# Autodesk Inventor assembly: ASY PNS 1200 right module
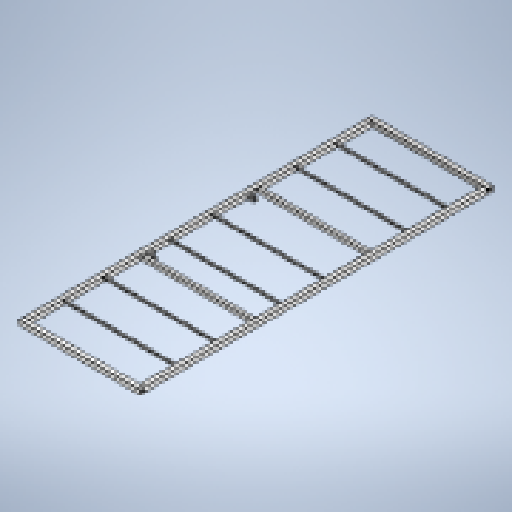
[picture p0: Inventor's stored thumbnail of the model, 512x512]
Saved by Autodesk Inventor 2025.3 (Build 293356030, 356C)
## iProperties
Created: 2025-03-25
Part Number: ASY PNS 1200 right module
Document SubType Name: Assembly
Designer: user
Author: user
## Documents named in this file (17)
- C:\Users\admin\Yandex.Disk\home pc\Inventor\PNS2-Panaevsk\ASY PNS 1200 right module.iam
- C:\Users\admin\Yandex.Disk\home pc\Inventor\PNS2-Panaevsk\ASY PNS 1220 frame right floor.iam
- C:\Users\admin\Yandex.Disk\home pc\Inventor\PNS2-Panaevsk\ASY PNS 1240 frame featheredge.iam
- C:\Users\admin\Yandex.Disk\home pc\Inventor\PNS2-Panaevsk\ASY PNS 1130 frame featheredge.iam
- C:\Users\admin\Yandex.Disk\home pc\Inventor\PNS2-Panaevsk\PNS-0261 Upper beam.ipt
- C:\Users\admin\Yandex.Disk\home pc\Inventor\PNS2-Panaevsk\PNS-0262 middle pillar.ipt
- C:\Users\admin\Yandex.Disk\home pc\Inventor\PNS2-Panaevsk\PNS-0262 cross beam.ipt
- C:\Users\admin\Yandex.Disk\home pc\Inventor\PNS2-Panaevsk\PNS-071 stretch ring.ipt
- C:\Users\admin\Yandex.Disk\home pc\Inventor\PNS2-Panaevsk\PNS-0310 strench.ipt
- C:\Users\admin\Yandex.Disk\home pc\Inventor\PNS2-Panaevsk\PNS-0810 floor ring.ipt
- C:\Users\admin\Yandex.Disk\home pc\Inventor\PNS2-Panaevsk\PNS-0812 floor ring  strengthen.ipt
- C:\Users\admin\Yandex.Disk\home pc\Inventor\PNS2-Panaevsk\PNS-073 stretch tear.ipt
- C:\Users\admin\Yandex.Disk\home pc\Inventor\PNS2-Panaevsk\PNS-0872 roof ring.ipt
- C:\Users\admin\Yandex.Disk\home pc\Inventor\PNS2-Panaevsk\PNS-077 stretch plate.ipt
- C:\Users\admin\Yandex.Disk\home pc\Inventor\PNS2-Panaevsk\PNS-0263 cross beam3.ipt
- C:\Users\admin\Yandex.Disk\home pc\Inventor\PNS2-Panaevsk\PNS-slings.ipt
- C:\Users\admin\Yandex.Disk\home pc\Inventor\PNS2-Panaevsk\PNS-slings_2.ipt
## Components (40 placed, 16 different names)
1. ASY PNS 1220 frame right floor:1 [sub-assembly] — Rigid:3, Mate:38, Flush:9, Mate:42, Mate:44, Mate:64, Mate:65, Mate:69
2. ASY PNS 1240 frame featheredge:1 [sub-assembly] — Rigid:4, Rigid:5, Rigid:6, Rigid:7, Mate:41, Mate:68
3. ASY PNS 1130 frame featheredge:1 [sub-assembly] — Rigid:3, Rigid:8, Rigid:9, Mate:37, Mate:40, Mate:55, Mate:56
4. PNS-0261 Upper beam:1 — Rigid:4, Mate:5, Flush:3, Mate:6, Flush:4, Mate:26, Mate:27, Tangent:4, Mate:35, Flush:8, Mate:39, Mate:46, Mate:49, Mate:50, Mate:51, Mate:52, Mate:53, Mate:54, Flush:17, Flush:18, Flush:19, Flush:20, Flush:21, Flush:22, Mate:61, Mate:63, Mate:67, Mate:77, Flush:73
5. PNS-0261 Upper beam:2 — Rigid:5, Mate:73, Mate:74, Mate:75, Mate:76
6. PNS-0262 middle pillar:1 — Rigid:6, Mate:43, Mate:66
7. PNS-0262 middle pillar:2 — Rigid:7, Flush:16
8. PNS-0262 middle pillar:3 — Rigid:8, Mate:36, Mate:45
9. PNS-0262 middle pillar:4 — Rigid:9, Flush:23
10. PNS-0262 cross beam:1 — Mate:6, Flush:4, Flush:23, Mate:57, Mate:58
11. PNS-0262 cross beam:2 — Mate:5, Flush:3, Flush:16, Mate:59, Mate:60
12. PNS-071 stretch ring:1 — Flush:12, Mate:66, Mate:67
13. PNS-071 stretch ring:2 — Flush:14, Mate:68, Mate:69
14. PNS-0310 strench:1
15. PNS-071 stretch ring:3 — Rotational:1, Mate:35, Mate:36, Flush:8, Flush:11, Flush:12
16. PNS-071 stretch ring:4 — Mate:37, Mate:38, Flush:9, Flush:10, Flush:14, Flush:15
17. PNS-0310 strench:2 — Mate:16, Tangent:3, Mate:17, Mate:21
18. PNS-0810 floor ring:2 — Mate:62, Flush:64, Flush:65, Mate:64
19. PNS-073 stretch tear:1 — Rotational:1, Mate:16, Tangent:3, Mate:17, Flush:6, Flush:7
20. PNS-073 stretch tear:2 — Mate:21, Flush:6, Flush:7
21. PNS-0812 floor ring  strengthen:2 — Mate:61, Mate:62, Flush:64, Flush:65, Mate:63, Flush:72
22. PNS-0810 floor ring:3 — Mate:28, Tangent:4
23. PNS-0812 floor ring  strengthen:3 — Mate:26, Mate:27, Mate:28, Mate:65, Flush:71
24. PNS-0872 roof ring:1 — Mate:77, Flush:73
25. PNS-077 stretch plate:1 — Mate:39, Mate:40, Flush:10
26. PNS-077 stretch plate:2 — Mate:44, Mate:45, Flush:11, Flush:13
27. PNS-077 stretch plate:3 — Mate:42, Mate:43, Flush:13
28. PNS-077 stretch plate:4 — Mate:41, Flush:15, Mate:46
29. PNS-0263 cross beam3:1 — Mate:49, Flush:22, Mate:55
30. PNS-0263 cross beam3:2 — Mate:50, Flush:21, Mate:56
31. PNS-0263 cross beam3:3 — Mate:51, Flush:20, Mate:57
32. PNS-0263 cross beam3:4 — Mate:52, Flush:19, Mate:58
33. PNS-0263 cross beam3:5 — Mate:53, Flush:18, Mate:59
34. PNS-0263 cross beam3:6 — Mate:54, Flush:17, Mate:60
35. PNS-slings:1
36. PNS-slings_2:1 — Mate:70
37. PNS-0810 floor ring:4
38. PNS-0812 floor ring  strengthen:4 — Mate:74, Mate:75, Flush:72
39. PNS-0810 floor ring:5
40. PNS-0812 floor ring  strengthen:5 — Mate:73, Mate:76, Flush:71
## Relationships (93: Mate 51, Flush 31, WeldJoint 8, Tangent 2, RevoluteJoint 1)
- [WeldJoint]: ASY PNS 1220 frame right floor:1 ↔ ASY PNS 1240 frame featheredge:1
- Rigid:3 [WeldJoint]: ASY PNS 1220 frame right floor:1 ↔ ASY PNS 1130 frame featheredge:1
- Rigid:4 [WeldJoint] (-100 mm): ASY PNS 1240 frame featheredge:1 ↔ PNS-0261 Upper beam:1
- Rigid:5 [WeldJoint] (-100 mm): ASY PNS 1240 frame featheredge:1 ↔ PNS-0261 Upper beam:2
- Rigid:6 [WeldJoint] (2200 mm): ASY PNS 1240 frame featheredge:1 ↔ PNS-0262 middle pillar:1
- Rigid:7 [WeldJoint] (2200 mm): ASY PNS 1240 frame featheredge:1 ↔ PNS-0262 middle pillar:2
- Rigid:8 [WeldJoint] (2200 mm): ASY PNS 1130 frame featheredge:1 ↔ PNS-0262 middle pillar:3
- Rigid:9 [WeldJoint] (2200 mm): ASY PNS 1130 frame featheredge:1 ↔ PNS-0262 middle pillar:4
- [Mate]: PNS-071 stretch ring:1 ↔ PNS-0310 strench:1
- [Flush]: PNS-071 stretch ring:1 ↔ PNS-0310 strench:1
- Mate:5: PNS-0261 Upper beam:1 ↔ PNS-0262 cross beam:2
- Flush:3: PNS-0261 Upper beam:1 ↔ PNS-0262 cross beam:2
- Mate:6: PNS-0261 Upper beam:1 ↔ PNS-0262 cross beam:1
- Flush:4: PNS-0261 Upper beam:1 ↔ PNS-0262 cross beam:1
- Rotational:1 [RevoluteJoint]: PNS-071 stretch ring:3 ↔ PNS-073 stretch tear:1
- Mate:16 (-50 mm): PNS-0310 strench:2 ↔ PNS-073 stretch tear:1
- Tangent:3: PNS-0310 strench:2 ↔ PNS-073 stretch tear:1
- Mate:17: PNS-0310 strench:2 ↔ PNS-073 stretch tear:1
- Mate:21 (-50 mm): PNS-0310 strench:2 ↔ PNS-073 stretch tear:2
- Flush:6: PNS-073 stretch tear:1 ↔ PNS-073 stretch tear:2
- Flush:7: PNS-073 stretch tear:1 ↔ PNS-073 stretch tear:2
- [Mate]: PNS-0810 floor ring:3 ↔ PNS-0812 floor ring  strengthen:3
- Mate:26: PNS-0261 Upper beam:1 ↔ PNS-0812 floor ring  strengthen:3
- Mate:27: PNS-0261 Upper beam:1 ↔ PNS-0812 floor ring  strengthen:3
- Mate:28: PNS-0810 floor ring:3 ↔ PNS-0812 floor ring  strengthen:3
- Tangent:4 (20 mm): PNS-0261 Upper beam:1 ↔ PNS-0810 floor ring:3
- Mate:35: PNS-0261 Upper beam:1 ↔ PNS-071 stretch ring:3
- Mate:36: PNS-0262 middle pillar:3 ↔ PNS-071 stretch ring:3
- Flush:8 (-50 mm): PNS-0261 Upper beam:1 ↔ PNS-071 stretch ring:3
- Mate:37: ASY PNS 1130 frame featheredge:1 ↔ PNS-071 stretch ring:4
- Mate:38: ASY PNS 1220 frame right floor:1 ↔ PNS-071 stretch ring:4
- Flush:9 (50 mm): ASY PNS 1220 frame right floor:1 ↔ PNS-071 stretch ring:4
- Mate:39: PNS-0261 Upper beam:1 ↔ PNS-077 stretch plate:1
- Mate:40: ASY PNS 1130 frame featheredge:1 ↔ PNS-077 stretch plate:1
- Flush:10: PNS-071 stretch ring:4 ↔ PNS-077 stretch plate:1
- Mate:41: ASY PNS 1240 frame featheredge:1 ↔ PNS-077 stretch plate:4
- Mate:42: ASY PNS 1220 frame right floor:1 ↔ PNS-077 stretch plate:3
- Mate:43: PNS-0262 middle pillar:1 ↔ PNS-077 stretch plate:3
- Mate:44: ASY PNS 1220 frame right floor:1 ↔ PNS-077 stretch plate:2
- Mate:45: PNS-0262 middle pillar:3 ↔ PNS-077 stretch plate:2
- Flush:11: PNS-071 stretch ring:3 ↔ PNS-077 stretch plate:2
- Flush:12: PNS-071 stretch ring:1 ↔ PNS-071 stretch ring:3
- Flush:13: PNS-077 stretch plate:2 ↔ PNS-077 stretch plate:3
- Flush:14: PNS-071 stretch ring:2 ↔ PNS-071 stretch ring:4
- Flush:15: PNS-071 stretch ring:4 ↔ PNS-077 stretch plate:4
- Mate:46: PNS-0261 Upper beam:1 ↔ PNS-077 stretch plate:4
- Flush:16 (-10 mm): PNS-0262 middle pillar:2 ↔ PNS-0262 cross beam:2
- Mate:49: PNS-0261 Upper beam:1 ↔ PNS-0263 cross beam3:1
- Mate:50: PNS-0261 Upper beam:1 ↔ PNS-0263 cross beam3:2
- Mate:51: PNS-0261 Upper beam:1 ↔ PNS-0263 cross beam3:3
- Mate:52: PNS-0261 Upper beam:1 ↔ PNS-0263 cross beam3:4
- Mate:53: PNS-0261 Upper beam:1 ↔ PNS-0263 cross beam3:5
- Mate:54: PNS-0261 Upper beam:1 ↔ PNS-0263 cross beam3:6
- Flush:17: PNS-0261 Upper beam:1 ↔ PNS-0263 cross beam3:6
- Flush:18: PNS-0261 Upper beam:1 ↔ PNS-0263 cross beam3:5
- Flush:19: PNS-0261 Upper beam:1 ↔ PNS-0263 cross beam3:4
- Flush:20: PNS-0261 Upper beam:1 ↔ PNS-0263 cross beam3:3
- Flush:21: PNS-0261 Upper beam:1 ↔ PNS-0263 cross beam3:2
- Flush:22: PNS-0261 Upper beam:1 ↔ PNS-0263 cross beam3:1
- Flush:23 (10 mm): PNS-0262 middle pillar:4 ↔ PNS-0262 cross beam:1
- Mate:55 (700 mm): ASY PNS 1130 frame featheredge:1 ↔ PNS-0263 cross beam3:1
- Mate:56 (1500 mm): ASY PNS 1130 frame featheredge:1 ↔ PNS-0263 cross beam3:2
- Mate:57 (850 mm): PNS-0262 cross beam:1 ↔ PNS-0263 cross beam3:3
- Mate:58 (1700 mm): PNS-0262 cross beam:1 ↔ PNS-0263 cross beam3:4
- Mate:59 (700 mm): PNS-0262 cross beam:2 ↔ PNS-0263 cross beam3:5
- Mate:60 (1500 mm): PNS-0262 cross beam:2 ↔ PNS-0263 cross beam3:6
- Mate:61: PNS-0261 Upper beam:1 ↔ PNS-0812 floor ring  strengthen:2
- Mate:62: PNS-0810 floor ring:2 ↔ PNS-0812 floor ring  strengthen:2
- Flush:64: PNS-0810 floor ring:2 ↔ PNS-0812 floor ring  strengthen:2
- Flush:65 (20 mm): PNS-0810 floor ring:2 ↔ PNS-0812 floor ring  strengthen:2
- Mate:63: PNS-0261 Upper beam:1 ↔ PNS-0812 floor ring  strengthen:2
- Mate:64: ASY PNS 1220 frame right floor:1 ↔ PNS-0810 floor ring:2
- Mate:65: ASY PNS 1220 frame right floor:1 ↔ PNS-0812 floor ring  strengthen:3
- Mate:66: PNS-0262 middle pillar:1 ↔ PNS-071 stretch ring:1
- Mate:67: PNS-0261 Upper beam:1 ↔ PNS-071 stretch ring:1
- Mate:68: ASY PNS 1240 frame featheredge:1 ↔ PNS-071 stretch ring:2
- Mate:69: ASY PNS 1220 frame right floor:1 ↔ PNS-071 stretch ring:2
- [Flush]: PNS-slings:1
- Mate:70: PNS-slings_2:1
- [Mate]: PNS-0810 floor ring:4 ↔ PNS-0812 floor ring  strengthen:4
- [Flush]: PNS-0810 floor ring:4 ↔ PNS-0812 floor ring  strengthen:4
- [Flush] (20 mm): PNS-0810 floor ring:4 ↔ PNS-0812 floor ring  strengthen:4
- [Mate]: PNS-0810 floor ring:5 ↔ PNS-0812 floor ring  strengthen:5
- [Flush]: PNS-0810 floor ring:5 ↔ PNS-0812 floor ring  strengthen:5
- [Flush] (20 mm): PNS-0810 floor ring:5 ↔ PNS-0812 floor ring  strengthen:5
- Mate:73: PNS-0261 Upper beam:2 ↔ PNS-0812 floor ring  strengthen:5
- Mate:74: PNS-0261 Upper beam:2 ↔ PNS-0812 floor ring  strengthen:4
- Mate:75: PNS-0261 Upper beam:2 ↔ PNS-0812 floor ring  strengthen:4
- Mate:76: PNS-0261 Upper beam:2 ↔ PNS-0812 floor ring  strengthen:5
- Flush:71: PNS-0812 floor ring  strengthen:3 ↔ PNS-0812 floor ring  strengthen:5
- Flush:72: PNS-0812 floor ring  strengthen:2 ↔ PNS-0812 floor ring  strengthen:4
- Mate:77: PNS-0261 Upper beam:1 ↔ PNS-0872 roof ring:1
- Flush:73 (10 mm): PNS-0261 Upper beam:1 ↔ PNS-0872 roof ring:1
## Named parameters: d18_d19 = 0 mm, d63_d62 = 0 mm, d146_d132 = 0 mm, d147_d133 = 0 mm, d148_d134 = 20 mm, d149_d132 = 0 mm, d150_d133 = 0 mm, d151_d134 = 20 mm
